# Autodesk Inventor assembly: liftidea1
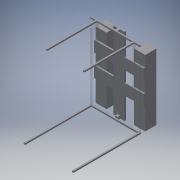
[picture p0: Inventor's stored thumbnail of the model, 180x180]
Saved by Autodesk Inventor 2017 (Build 210142000, 142)
## iProperties
Created: 2017-05-30
Part Number: liftidea1
Document SubType Name: Assembly
Designer: User
Author: User
## Documents named in this file (7)
- C:\Robotics\CAD\2016-17_CAD\liftidea1.iam
- C:\Robotics\CAD\2016-17_CAD\topbarlift.ipt
- C:\Robotics\CAD\2016-17_CAD\backplatelift.ipt
- C:\Robotics\CAD\2016-17_CAD\bottombarlift.ipt
- C:\Robotics\CAD\2016-17_CAD\bottombarliftconnector.ipt
- C:\Robotics\CAD\2016-17_CAD\halfinchspacer.ipt
- C:\Robotics\CAD\2016-17_CAD\outlineslides.ipt
## Components (15 placed, 6 different names)
1. topbarlift:1 — Mate:1, Flush:1, Flush:2, Flush:27
2. topbarlift:2 — Mate:2, Flush:3, Flush:4, Flush:30
3. backplatelift:1 — Flush:5, Flush:7, Mate:7, Flush:13, Flush:14, Mate:9, Flush:15, Flush:16, Mate:11, Flush:17, Flush:18, Mate:12, Flush:19, Flush:20, Flush:21, Flush:22
4. bottombarlift:1 — Mate:6, Flush:11, Flush:12
5. bottombarlift:2 — Mate:5, Flush:9, Flush:10
6. topbarlift:3 — Mate:1, Flush:1, Flush:2, Mate:2, Flush:3, Flush:4, Flush:5, Mate:8, Flush:21, Mate:15, Flush:28, Mate:16, Flush:29
7. bottombarliftconnector:1 — Flush:7, Mate:5, Flush:9, Flush:10, Mate:6, Flush:11, Flush:12, Mate:10, Flush:22, Mate:13, Flush:23, Flush:24, Mate:14, Flush:25, Flush:26
8. halfinchspacer:1 — Mate:9, Flush:15, Mate:10, Flush:16
9. halfinchspacer:2 — Mate:7, Flush:13, Mate:8, Flush:14
10. outlineslides:1 — Mate:11, Flush:17, Flush:18
11. outlineslides:2 — Mate:12, Flush:19, Flush:20
12. bottombarlift:3 — Mate:14, Flush:25, Flush:26
13. bottombarlift:4 — Mate:13, Flush:23, Flush:24
14. topbarlift:4 — Mate:15, Flush:27, Flush:28
15. topbarlift:5 — Mate:16, Flush:29, Flush:30
## Relationships (42: Flush 28, Mate 14)
- Mate:1: topbarlift:1 ↔ topbarlift:3
- Flush:1 (-25.4 mm): topbarlift:1 ↔ topbarlift:3
- Flush:2: topbarlift:1 ↔ topbarlift:3
- Mate:2: topbarlift:2 ↔ topbarlift:3
- Flush:3 (25.4 mm): topbarlift:2 ↔ topbarlift:3
- Flush:4: topbarlift:2 ↔ topbarlift:3
- Flush:5: backplatelift:1 ↔ topbarlift:3
- Flush:7: backplatelift:1 ↔ bottombarliftconnector:1
- Mate:5: bottombarlift:2 ↔ bottombarliftconnector:1
- Flush:9: bottombarlift:2 ↔ bottombarliftconnector:1
- Flush:10: bottombarlift:2 ↔ bottombarliftconnector:1
- Mate:6: bottombarlift:1 ↔ bottombarliftconnector:1
- Flush:11: bottombarlift:1 ↔ bottombarliftconnector:1
- Flush:12: bottombarlift:1 ↔ bottombarliftconnector:1
- Mate:7: backplatelift:1 ↔ halfinchspacer:2
- Flush:13: backplatelift:1 ↔ halfinchspacer:2
- Mate:8: topbarlift:3 ↔ halfinchspacer:2
- Flush:14 (19.05 mm): backplatelift:1 ↔ halfinchspacer:2
- Mate:9: backplatelift:1 ↔ halfinchspacer:1
- Flush:15: backplatelift:1 ↔ halfinchspacer:1
- Mate:10: bottombarliftconnector:1 ↔ halfinchspacer:1
- Flush:16 (19.05 mm): backplatelift:1 ↔ halfinchspacer:1
- Mate:11: backplatelift:1 ↔ outlineslides:1
- Flush:17: backplatelift:1 ↔ outlineslides:1
- Flush:18: backplatelift:1 ↔ outlineslides:1
- Mate:12: backplatelift:1 ↔ outlineslides:2
- Flush:19: backplatelift:1 ↔ outlineslides:2
- Flush:20: backplatelift:1 ↔ outlineslides:2
- Flush:21 (88.9 mm): backplatelift:1 ↔ topbarlift:3
- Flush:22 (88.9 mm): backplatelift:1 ↔ bottombarliftconnector:1
- Mate:13: bottombarliftconnector:1 ↔ bottombarlift:4
- Flush:23: bottombarliftconnector:1 ↔ bottombarlift:4
- Flush:24: bottombarliftconnector:1 ↔ bottombarlift:4
- Mate:14: bottombarliftconnector:1 ↔ bottombarlift:3
- Flush:25: bottombarliftconnector:1 ↔ bottombarlift:3
- Flush:26: bottombarliftconnector:1 ↔ bottombarlift:3
- Mate:15: topbarlift:3 ↔ topbarlift:4
- Flush:27: topbarlift:1 ↔ topbarlift:4
- Flush:28: topbarlift:3 ↔ topbarlift:4
- Mate:16: topbarlift:3 ↔ topbarlift:5
- Flush:29: topbarlift:3 ↔ topbarlift:5
- Flush:30: topbarlift:2 ↔ topbarlift:5
